# Autodesk Inventor assembly: Assy_fore_arm
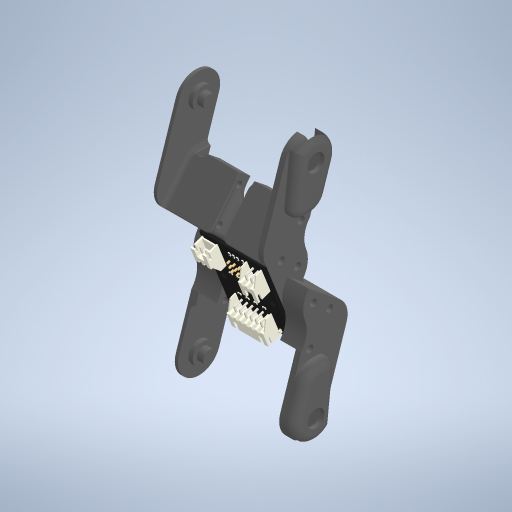
[picture p0: Inventor's stored thumbnail of the model, 512x512]
Saved by Autodesk Inventor 2024.1 (Build 281209000, 209)
## iProperties
Created: 2025-03-03
Part Number: Assy_fore_arm
Document SubType Name: Assembly
Designer: hibik
Author: hibik
## Documents named in this file (5)
- C:\Users\hibik\Documents\Robomech\RESCUE\ORCA\hard\arm\Assy_fore_arm.iam
- C:\Users\hibik\Documents\Robomech\RESCUE\ORCA\hard\arm\fore_arm_base.ipt
- C:\Users\hibik\Documents\Robomech\RESCUE\ORCA\hard\arm\fore_arm_side_left.ipt
- C:\Users\hibik\Documents\Robomech\RESCUE\ORCA\hard\arm\fore_arm_side_right.ipt
- C:\Users\hibik\Documents\Robomech\RESCUE\ORCA\hard\board\CORE_model\arm.iam
## Components (6 placed, 4 different names)
1. fore_arm_side_left:1 — 挿入:1, 挿入:2
2. fore_arm_side_right:1 — 挿入:3, 挿入:4, メイト:3
3. fore_arm_base:1 — 挿入:1, 挿入:2, 挿入:3, 挿入:4, 挿入:5, 挿入:6, 挿入:7, 挿入:8, メイト:1, 挿入:9, 角度:1, フラッシュ:1
4. fore_arm_side_left:2 — 挿入:7, 挿入:8
5. fore_arm_side_right:2 — 挿入:5, 挿入:6, メイト:2
6. arm:1 [sub-assembly] — メイト:1, 挿入:9, 角度:1
## Relationships (14: Insert 9, Mate 3, Angle 1, Flush 1)
- 挿入:1 [Insert]: fore_arm_side_left:1 ↔ fore_arm_base:1
- 挿入:2 [Insert]: fore_arm_side_left:1 ↔ fore_arm_base:1
- 挿入:3 [Insert]: fore_arm_side_right:1 ↔ fore_arm_base:1
- 挿入:4 [Insert]: fore_arm_side_right:1 ↔ fore_arm_base:1
- 挿入:5 [Insert]: fore_arm_base:1 ↔ fore_arm_side_right:2
- 挿入:6 [Insert]: fore_arm_base:1 ↔ fore_arm_side_right:2
- 挿入:7 [Insert]: fore_arm_base:1 ↔ fore_arm_side_left:2
- 挿入:8 [Insert]: fore_arm_base:1 ↔ fore_arm_side_left:2
- メイト:1 [Mate]: fore_arm_base:1 ↔ arm:1
- 挿入:9 [Insert]: fore_arm_base:1 ↔ arm:1
- 角度:1 [Angle] (0 deg): fore_arm_base:1 ↔ arm:1
- メイト:2 [Mate]: fore_arm_side_right:2
- フラッシュ:1 [Flush]: fore_arm_base:1
- メイト:3 [Mate]: fore_arm_side_right:1
